# Autodesk Inventor assembly: GearSet 1
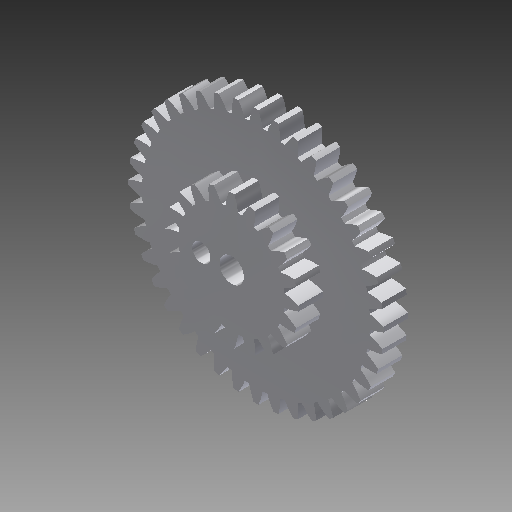
[picture p0: Inventor's stored thumbnail of the model, 512x512]
Saved by Autodesk Inventor 2017 SP1 (Build 210196100, 196)
## iProperties
Created: 2017-09-23
Part Number: GearSet 1
Document SubType Name: Assembly
Designer: Zach
Author: Zach
## Documents named in this file (3)
- C:\Users\Zach\Documents\GitHub\tr1\lib\Gearbox 128;1\GearSet 1.iam
- C:\Users\Zach\Documents\GitHub\tr1\lib\Gearbox 128;1\Design Accelerator\Spur Gear12.ipt
- C:\Users\Zach\Documents\GitHub\tr1\lib\Gearbox 128;1\Design Accelerator\Spur Gear22.ipt
## Components (2 placed, 2 different names)
1. Spur Gear1:1 — Mate:1, Mate:2, Mate:3
2. Spur Gear2:1 — Mate:1, Mate:2, Mate:3
## Relationships (3: Mate 3)
- Mate:1: Spur Gear1:1 ↔ Spur Gear2:1
- Mate:2: Spur Gear1:1 ↔ Spur Gear2:1
- Mate:3: Spur Gear1:1 ↔ Spur Gear2:1
